# Autodesk Inventor assembly: calosc
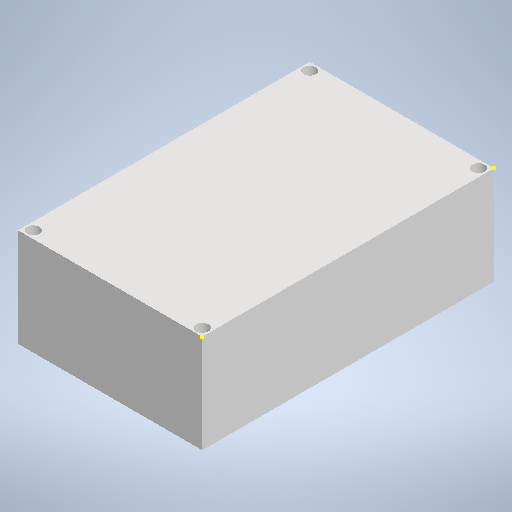
[picture p0: Inventor's stored thumbnail of the model, 512x512]
Saved by Autodesk Inventor 2025 (Build 290162000, 162)
## iProperties
Created: 2024-12-22
Part Number: calosc
Document SubType Name: Assembly
Designer: Admin
Author: Admin
## Documents named in this file (3)
- C:\Studia\Semestr_7\inzynierka\calosc.iam
- C:\Studia\Semestr_7\inzynierka\dol.ipt
- C:\Studia\Semestr_7\inzynierka\góra.ipt
## Components (2 placed, 2 different names)
1. dol:1 — Sztywne:1
2. góra:1 — Sztywne:1
## Relationships (1: WeldJoint 1)
- Sztywne:1 [WeldJoint]: dol:1 ↔ góra:1
